# Autodesk Inventor assembly: Manipulator
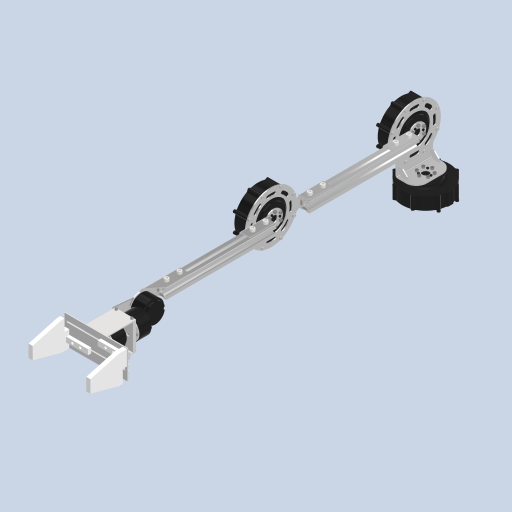
[picture p0: Inventor's stored thumbnail of the model, 512x512]
Saved by Autodesk Inventor 2023 (Build 270158000, 158)
## iProperties
Created: 2024-11-08
Part Number: Manipulator
Document SubType Name: Assembly
Designer: kiyo
Author: kiyo
## Documents named in this file (19)
- D:\GitHub\inventor\syu-si\OfficeRobot\Manipulator\Manipulator.iam
- D:\GitHub\inventor\syu-si\OfficeRobot\ReadyMade\Steadywin\GIM8108-8.iam
- D:\GitHub\inventor\syu-si\OfficeRobot\Manipulator\elbow-pitch-bracket.ipt
- D:\GitHub\inventor\syu-si\OfficeRobot\ReadyMade\Screw\M3_6mm.ipt
- D:\GitHub\inventor\syu-si\OfficeRobot\ReadyMade\Steadywin\GIM3505-8_with-driver.ipt
- D:\GitHub\inventor\syu-si\OfficeRobot\Manipulator\wrist_roll_plate.ipt
- D:\GitHub\inventor\syu-si\OfficeRobot\Manipulator\wrist-pitch-plate.ipt
- D:\GitHub\inventor\syu-si\OfficeRobot\ReadyMade\Screw\M2-5_6mm.ipt
- D:\GitHub\inventor\syu-si\OfficeRobot\ReadyMade\Screw\CBSH3-8.ipt
- D:\GitHub\inventor\syu-si\OfficeRobot\ReadyMade\Screw\FWSJJ-D5-V2_6-T4_5.ipt
- D:\GitHub\inventor\syu-si\OfficeRobot\ReadyMade\Screw\M2-5_10mm.ipt
- D:\GitHub\inventor\syu-si\OfficeRobot\ReadyMade\Screw\HNTU5-5.ipt
- D:\GitHub\inventor\syu-si\OfficeRobot\Manipulator\pitch_plate_20mm.ipt
- D:\GitHub\inventor\syu-si\OfficeRobot\ReadyMade\Aluminum-frame\HFS5-2020-210-AV10-BV35-CV175-DV200.ipt
- D:\GitHub\inventor\syu-si\OfficeRobot\Manipulator\sholder_roll_bracket.ipt
- D:\GitHub\inventor\syu-si\OfficeRobot\ReadyMade\Screw\SCB5-22.ipt
- D:\GitHub\inventor\syu-si\OfficeRobot\ReadyMade\Screw\SCB5-8.ipt
- D:\GitHub\inventor\syu-si\OfficeRobot\Manipulator\Hand_tyokudou.iam
- D:\GitHub\inventor\syu-si\OfficeRobot\ReadyMade\Screw\PACK-SWSJJ10-6-0_3.ipt
## Components (110 placed, 18 different names)
1. pitch_plate_20mm:1 — メイト:3, フラッシュ:1, 挿入:355, 挿入:356, 挿入:357, 挿入:358, 挿入:359, 挿入:360, 角度:47
2. pitch_plate_20mm:2 — 挿入:345, フラッシュ:3, 角度:40
3. elbow-pitch-bracket:1 — 挿入:341, 挿入:342, フラッシュ:2, フラッシュ:7, フラッシュ:8
4. sholder_roll_bracket:1 — 挿入:350, 挿入:361, 挿入:362, 挿入:363, 挿入:364, 挿入:365, 挿入:366, 挿入:414, 挿入:415
5. HFS5-2020-210-AV10-BV35-CV175-DV200:1 — メイト:3, フラッシュ:1, フラッシュ:2, メイト:19, メイト:20, 角度:35, 角度:36, メイト:21, メイト:22, フラッシュ:9, 角度:37, メイト:23, メイト:24
6. HFS5-2020-210-AV10-BV35-CV175-DV200:2 — フラッシュ:3, 挿入:351, 挿入:352, 角度:27, 角度:28, 挿入:353, 挿入:354, 角度:29, 角度:30, メイト:15, メイト:16, 角度:33, フラッシュ:5, メイト:17, メイト:18, 角度:34, フラッシュ:6, メイト:25, メイト:26, メイト:27, メイト:28, メイト:29, メイト:30
7. wrist-pitch-plate:1 — 挿入:409, 挿入:410, メイト:29, メイト:30, 正接:1, 正接:2, 正接:3, 挿入:437, 挿入:438, 挿入:439
8. wrist_roll_plate:2 — 挿入:402, 挿入:403, 挿入:404, 挿入:405, 挿入:406, 挿入:407, 挿入:408
9. Hand_tyokudou:1 [sub-assembly] — 角度:45, 挿入:431, 挿入:434, 挿入:435, 挿入:436
10. PACK-SWSJJ10-6-0_3:1 — 挿入:429
11. PACK-SWSJJ10-6-0_3:2 — 挿入:428
12. PACK-SWSJJ10-6-0_3:3 — 挿入:418
13. PACK-SWSJJ10-6-0_3:4 — 挿入:419
14. PACK-SWSJJ10-6-0_3:5 — 挿入:421
15. PACK-SWSJJ10-6-0_3:6 — 挿入:426
16. PACK-SWSJJ10-6-0_3:7 — 挿入:423
17. PACK-SWSJJ10-6-0_3:8 — 挿入:424
18. PACK-SWSJJ10-6-0_3:9 — 挿入:422
19. PACK-SWSJJ10-6-0_3:10 — 挿入:425
20. PACK-SWSJJ10-6-0_3:11 — 挿入:420
21. PACK-SWSJJ10-6-0_3:12 — 挿入:427
22. PACK-SWSJJ10-6-0_3:13 — 挿入:417
23. PACK-SWSJJ10-6-0_3:14 — 挿入:416
24. FWSJJ-D5-V2_6-T4_5:13 — 挿入:430, 挿入:431
25. M2-5_10mm:10 — 挿入:430
26. FWSJJ-D5-V2_6-T4_5:14 — 挿入:434
27. M2-5_10mm:11
28. FWSJJ-D5-V2_6-T4_5:15 — 挿入:435
29. M2-5_10mm:12
30. M2-5_6mm:16 — 挿入:439
31. M2-5_6mm:17 — 挿入:438
32. M2-5_6mm:18 — 挿入:437
33. M3_6mm:7 — 挿入:337
34. M3_6mm:8 — 挿入:336
35. M3_6mm:9 — 挿入:334
36. M3_6mm:10 — 挿入:338
37. M3_6mm:11 — 挿入:339
38. M3_6mm:12 — 挿入:335
39. M3_6mm:19 — 挿入:358
40. M3_6mm:20 — 挿入:357
41. M3_6mm:21 — 挿入:355
42. M3_6mm:22 — 挿入:356
43. M3_6mm:23 — 挿入:359
44. M3_6mm:24 — 挿入:360
45. M3_6mm:25 — 挿入:361
46. M3_6mm:26 — 挿入:363
47. M3_6mm:27 — 挿入:362
48. M3_6mm:28 — 挿入:364
49. M3_6mm:29 — 挿入:365
50. M3_6mm:30 — 挿入:366
51. CBSH3-8:1 — 挿入:307
52. CBSH3-8:2 — 挿入:308
53. CBSH3-8:3 — 挿入:302
54. CBSH3-8:4 — 挿入:304, 挿入:415
55. CBSH3-8:5 — 挿入:309
56. CBSH3-8:6 — 挿入:303
57. CBSH3-8:7 — 挿入:305
58. CBSH3-8:8 — 挿入:306
59. CBSH3-8:9 — 挿入:332
60. CBSH3-8:10 — 挿入:327
61. CBSH3-8:11 — 挿入:330
62. CBSH3-8:12 — 挿入:328
63. CBSH3-8:13 — 挿入:329
64. CBSH3-8:14 — 挿入:331
65. CBSH3-8:15 — 挿入:326
66. CBSH3-8:16 — 挿入:333
67. M2-5_6mm:13
68. M2-5_6mm:14
69. M2-5_6mm:15
70. M2-5_10mm:7 — 挿入:402
71. M2-5_10mm:8 — 挿入:403
72. M2-5_10mm:9 — 挿入:404
73. FWSJJ-D5-V2_6-T4_5:10 — 挿入:407
74. FWSJJ-D5-V2_6-T4_5:11 — 挿入:405
75. FWSJJ-D5-V2_6-T4_5:12 — 挿入:406
76. HNTU5-5:22 — 挿入:412, メイト:27, メイト:28
77. SCB5-8:8 — 挿入:412, 正接:2, 挿入:429
78. HNTU5-5:23 — 挿入:411, メイト:25, メイト:26
79. SCB5-8:9 — 挿入:411, 正接:3, 挿入:428
80. SCB5-22:1 — 挿入:368, 挿入:418
81. SCB5-22:2 — 挿入:367, 挿入:419
82. SCB5-22:3 — 挿入:370, 挿入:421
83. SCB5-22:4 — 挿入:369, 挿入:420
84. SCB5-22:5 — 挿入:372, 挿入:423
85. SCB5-22:6 — 挿入:371, 挿入:422
86. SCB5-22:7 — 挿入:376, 挿入:416
87. SCB5-22:8 — 挿入:375, 正接:1, 挿入:417
88. SCB5-8:3 — 挿入:427
89. SCB5-8:4
90. SCB5-8:5 — 挿入:426
91. SCB5-8:6 — 挿入:425
92. SCB5-8:7 — 挿入:424
93. HNTU5-5:6 — 挿入:372
94. HNTU5-5:7 — 挿入:371
95. HNTU5-5:9 — 挿入:369
96. HNTU5-5:10 — 挿入:370
97. HNTU5-5:11 — 挿入:351, 角度:28, 挿入:367
98. HNTU5-5:12 — 挿入:352, 角度:27, 挿入:368
99. HNTU5-5:13 — 挿入:353, 角度:30, 挿入:376
100. HNTU5-5:14 — 挿入:354, 角度:29, 挿入:375
101. HNTU5-5:17 — メイト:15, メイト:16, 角度:33, フラッシュ:5
102. HNTU5-5:18 — メイト:17, メイト:18, 角度:34, フラッシュ:6
103. HNTU5-5:19 — フラッシュ:8, メイト:19, メイト:20, 角度:35
104. HNTU5-5:20 — フラッシュ:7, 角度:36, メイト:21, メイト:22
105. HNTU5-5:21 — フラッシュ:9, 角度:37, メイト:23, メイト:24
106. GIM8108-8:1 [sub-assembly] — 挿入:350, 角度:46, 角度:48
107. GIM8108-8:2 [sub-assembly] — 挿入:302, 挿入:303, 挿入:304, 挿入:305, 挿入:306, 挿入:307, 挿入:308, 挿入:309, 角度:46, 挿入:414, 角度:47
108. GIM8108-8:3 [sub-assembly] — 挿入:326, 挿入:327, 挿入:328, 挿入:329, 挿入:330, 挿入:331, 挿入:332, 挿入:333, 挿入:334, 挿入:335, 挿入:336, 挿入:337, 挿入:338, 挿入:339, 挿入:341, 挿入:342, 挿入:345, 角度:40
109. GIM3505-8_with-driver:9 — 挿入:408, 挿入:409, 挿入:410, 角度:44
110. GIM3505-8_with-driver:8 — 角度:44, 角度:45, 挿入:436
## Relationships (155: Insert 102, Mate 22, Angle 20, Flush 8, Tangent 3)
- 挿入:302 [Insert] (2 mm): CBSH3-8:3 ↔ GIM8108-8:2
- 挿入:303 [Insert] (2 mm): CBSH3-8:6 ↔ GIM8108-8:2
- 挿入:304 [Insert] (2 mm): CBSH3-8:4 ↔ GIM8108-8:2
- 挿入:305 [Insert] (2 mm): CBSH3-8:7 ↔ GIM8108-8:2
- 挿入:306 [Insert] (2 mm): CBSH3-8:8 ↔ GIM8108-8:2
- 挿入:307 [Insert] (2 mm): CBSH3-8:1 ↔ GIM8108-8:2
- 挿入:308 [Insert] (2 mm): CBSH3-8:2 ↔ GIM8108-8:2
- 挿入:309 [Insert] (2 mm): CBSH3-8:5 ↔ GIM8108-8:2
- [Insert] (-0.75 mm): HFS5-2020-210-AV10-BV35-CV175-DV200:1 ↔ HNTU5-5:6
- [Angle] (0 deg): HFS5-2020-210-AV10-BV35-CV175-DV200:1 ↔ HNTU5-5:6
- [Insert] (-0.75 mm): HFS5-2020-210-AV10-BV35-CV175-DV200:1 ↔ HNTU5-5:7
- [Angle] (0 deg): HFS5-2020-210-AV10-BV35-CV175-DV200:1 ↔ HNTU5-5:7
- [Angle] (0 deg): HFS5-2020-210-AV10-BV35-CV175-DV200:1 ↔ HNTU5-5:6
- 挿入:326 [Insert] (2 mm): CBSH3-8:15 ↔ GIM8108-8:3
- 挿入:327 [Insert] (2 mm): CBSH3-8:10 ↔ GIM8108-8:3
- 挿入:328 [Insert] (2 mm): CBSH3-8:12 ↔ GIM8108-8:3
- 挿入:329 [Insert] (2 mm): CBSH3-8:13 ↔ GIM8108-8:3
- 挿入:330 [Insert] (2 mm): CBSH3-8:11 ↔ GIM8108-8:3
- 挿入:331 [Insert] (2 mm): CBSH3-8:14 ↔ GIM8108-8:3
- 挿入:332 [Insert] (2 mm): CBSH3-8:9 ↔ GIM8108-8:3
- 挿入:333 [Insert] (2 mm): CBSH3-8:16 ↔ GIM8108-8:3
- 挿入:334 [Insert] (2 mm): M3_6mm:9 ↔ GIM8108-8:3
- 挿入:335 [Insert] (2 mm): M3_6mm:12 ↔ GIM8108-8:3
- 挿入:336 [Insert] (2 mm): M3_6mm:8 ↔ GIM8108-8:3
- 挿入:337 [Insert] (2 mm): M3_6mm:7 ↔ GIM8108-8:3
- 挿入:338 [Insert] (2 mm): M3_6mm:10 ↔ GIM8108-8:3
- 挿入:339 [Insert] (2 mm): M3_6mm:11 ↔ GIM8108-8:3
- [Insert]: pitch_plate_20mm:1 ↔ GIM8108-8:2
- [Mate] (0.3 mm): pitch_plate_20mm:1 ↔ HFS5-2020-210-AV10-BV35-CV175-DV200:1
- メイト:3 [Mate] (0.3 mm): pitch_plate_20mm:1 ↔ HFS5-2020-210-AV10-BV35-CV175-DV200:1
- 挿入:341 [Insert]: elbow-pitch-bracket:1 ↔ GIM8108-8:3
- 挿入:342 [Insert]: elbow-pitch-bracket:1 ↔ GIM8108-8:3
- [Angle] (0 deg): HFS5-2020-210-AV10-BV35-CV175-DV200:1 ↔ HNTU5-5:9
- [Angle] (0 deg): HFS5-2020-210-AV10-BV35-CV175-DV200:1 ↔ HNTU5-5:10
- [Insert] (-0.75 mm): HFS5-2020-210-AV10-BV35-CV175-DV200:1 ↔ HNTU5-5:9
- [Insert] (-0.75 mm): HFS5-2020-210-AV10-BV35-CV175-DV200:1 ↔ HNTU5-5:10
- [Mate] (0.3 mm): elbow-pitch-bracket:1 ↔ HFS5-2020-210-AV10-BV35-CV175-DV200:1
- [Mate] (0.3 mm): elbow-pitch-bracket:1 ↔ HFS5-2020-210-AV10-BV35-CV175-DV200:1
- 挿入:345 [Insert]: pitch_plate_20mm:2 ↔ GIM8108-8:3
- [Mate] (0.3 mm): pitch_plate_20mm:2 ↔ HFS5-2020-210-AV10-BV35-CV175-DV200:2
- [Mate] (0.3 mm): pitch_plate_20mm:2 ↔ HFS5-2020-210-AV10-BV35-CV175-DV200:2
- 挿入:350 [Insert]: sholder_roll_bracket:1 ↔ GIM8108-8:1
- フラッシュ:1 [Flush]: pitch_plate_20mm:1 ↔ HFS5-2020-210-AV10-BV35-CV175-DV200:1
- フラッシュ:2 [Flush]: elbow-pitch-bracket:1 ↔ HFS5-2020-210-AV10-BV35-CV175-DV200:1
- フラッシュ:3 [Flush]: pitch_plate_20mm:2 ↔ HFS5-2020-210-AV10-BV35-CV175-DV200:2
- 挿入:351 [Insert] (-0.75 mm): HFS5-2020-210-AV10-BV35-CV175-DV200:2 ↔ HNTU5-5:11
- 挿入:352 [Insert] (-0.75 mm): HFS5-2020-210-AV10-BV35-CV175-DV200:2 ↔ HNTU5-5:12
- 角度:27 [Angle] (0 deg): HFS5-2020-210-AV10-BV35-CV175-DV200:2 ↔ HNTU5-5:12
- 角度:28 [Angle] (0 deg): HFS5-2020-210-AV10-BV35-CV175-DV200:2 ↔ HNTU5-5:11
- 挿入:353 [Insert] (-0.75 mm): HFS5-2020-210-AV10-BV35-CV175-DV200:2 ↔ HNTU5-5:13
- 挿入:354 [Insert] (-0.75 mm): HFS5-2020-210-AV10-BV35-CV175-DV200:2 ↔ HNTU5-5:14
- 角度:29 [Angle] (0 deg): HFS5-2020-210-AV10-BV35-CV175-DV200:2 ↔ HNTU5-5:14
- 角度:30 [Angle] (0 deg): HFS5-2020-210-AV10-BV35-CV175-DV200:2 ↔ HNTU5-5:13
- 挿入:355 [Insert]: pitch_plate_20mm:1 ↔ M3_6mm:21
- 挿入:356 [Insert]: pitch_plate_20mm:1 ↔ M3_6mm:22
- 挿入:357 [Insert]: pitch_plate_20mm:1 ↔ M3_6mm:20
- 挿入:358 [Insert]: pitch_plate_20mm:1 ↔ M3_6mm:19
- 挿入:359 [Insert]: pitch_plate_20mm:1 ↔ M3_6mm:23
- 挿入:360 [Insert]: pitch_plate_20mm:1 ↔ M3_6mm:24
- 挿入:361 [Insert]: sholder_roll_bracket:1 ↔ M3_6mm:25
- 挿入:362 [Insert]: sholder_roll_bracket:1 ↔ M3_6mm:27
- 挿入:363 [Insert]: sholder_roll_bracket:1 ↔ M3_6mm:26
- 挿入:364 [Insert]: sholder_roll_bracket:1 ↔ M3_6mm:28
- 挿入:365 [Insert]: sholder_roll_bracket:1 ↔ M3_6mm:29
- 挿入:366 [Insert]: sholder_roll_bracket:1 ↔ M3_6mm:30
- 挿入:367 [Insert] (-0.95 mm): SCB5-22:2 ↔ HNTU5-5:11
- 挿入:368 [Insert] (-0.95 mm): SCB5-22:1 ↔ HNTU5-5:12
- 挿入:369 [Insert] (-0.95 mm): SCB5-22:4 ↔ HNTU5-5:9
- 挿入:370 [Insert] (-0.95 mm): SCB5-22:3 ↔ HNTU5-5:10
- 挿入:371 [Insert] (-0.95 mm): SCB5-22:6 ↔ HNTU5-5:7
- 挿入:372 [Insert] (-0.95 mm): SCB5-22:5 ↔ HNTU5-5:6
- 挿入:375 [Insert] (-0.95 mm): SCB5-22:8 ↔ HNTU5-5:14
- 挿入:376 [Insert] (-0.95 mm): SCB5-22:7 ↔ HNTU5-5:13
- [Insert] (3.5 mm): SCB5-8:3 ↔ HNTU5-5:17
- メイト:15 [Mate]: HFS5-2020-210-AV10-BV35-CV175-DV200:2 ↔ HNTU5-5:17
- メイト:16 [Mate] (1 mm): HFS5-2020-210-AV10-BV35-CV175-DV200:2 ↔ HNTU5-5:17
- 角度:33 [Angle] (0 deg): HFS5-2020-210-AV10-BV35-CV175-DV200:2 ↔ HNTU5-5:17
- フラッシュ:5 [Flush] (33.5 mm): HFS5-2020-210-AV10-BV35-CV175-DV200:2 ↔ HNTU5-5:17
- [Insert] (3.2 mm): SCB5-8:4 ↔ HNTU5-5:18
- メイト:17 [Mate]: HFS5-2020-210-AV10-BV35-CV175-DV200:2 ↔ HNTU5-5:18
- メイト:18 [Mate] (1 mm): HFS5-2020-210-AV10-BV35-CV175-DV200:2 ↔ HNTU5-5:18
- 角度:34 [Angle] (0 deg): HFS5-2020-210-AV10-BV35-CV175-DV200:2 ↔ HNTU5-5:18
- フラッシュ:6 [Flush] (33.5 mm): HFS5-2020-210-AV10-BV35-CV175-DV200:2 ↔ HNTU5-5:18
- [Insert] (3.5 mm): SCB5-8:5 ↔ HNTU5-5:19
- [Insert] (3.5 mm): SCB5-8:6 ↔ HNTU5-5:20
- フラッシュ:7 [Flush] (5.5 mm): elbow-pitch-bracket:1 ↔ HNTU5-5:20
- フラッシュ:8 [Flush] (-30.5 mm): elbow-pitch-bracket:1 ↔ HNTU5-5:19
- メイト:19 [Mate]: HFS5-2020-210-AV10-BV35-CV175-DV200:1 ↔ HNTU5-5:19
- メイト:20 [Mate] (1 mm): HFS5-2020-210-AV10-BV35-CV175-DV200:1 ↔ HNTU5-5:19
- 角度:35 [Angle] (0 deg): HFS5-2020-210-AV10-BV35-CV175-DV200:1 ↔ HNTU5-5:19
- 角度:36 [Angle] (0 deg): HFS5-2020-210-AV10-BV35-CV175-DV200:1 ↔ HNTU5-5:20
- メイト:21 [Mate] (1 mm): HFS5-2020-210-AV10-BV35-CV175-DV200:1 ↔ HNTU5-5:20
- メイト:22 [Mate]: HFS5-2020-210-AV10-BV35-CV175-DV200:1 ↔ HNTU5-5:20
- [Insert] (3.5 mm): SCB5-8:7 ↔ HNTU5-5:21
- フラッシュ:9 [Flush] (33.5 mm): HFS5-2020-210-AV10-BV35-CV175-DV200:1 ↔ HNTU5-5:21
- 角度:37 [Angle] (0 deg): HFS5-2020-210-AV10-BV35-CV175-DV200:1 ↔ HNTU5-5:21
- メイト:23 [Mate] (1 mm): HFS5-2020-210-AV10-BV35-CV175-DV200:1 ↔ HNTU5-5:21
- メイト:24 [Mate]: HFS5-2020-210-AV10-BV35-CV175-DV200:1 ↔ HNTU5-5:21
- 角度:40 [Angle] (0 deg): pitch_plate_20mm:2 ↔ GIM8108-8:3
- [Insert]: wrist_roll_plate:2 ↔ M2-5_6mm:13
- [Insert]: wrist_roll_plate:2 ↔ M2-5_6mm:14
- [Insert]: wrist_roll_plate:2 ↔ M2-5_6mm:15
- [Insert]: wrist_roll_plate:2 ↔ GIM3505-8_with-driver:8
- [Insert]: wrist_roll_plate:2 ↔ GIM3505-8_with-driver:8
- 挿入:402 [Insert]: wrist_roll_plate:2 ↔ M2-5_10mm:7
- 挿入:403 [Insert]: wrist_roll_plate:2 ↔ M2-5_10mm:8
- 挿入:404 [Insert]: wrist_roll_plate:2 ↔ M2-5_10mm:9
- 挿入:405 [Insert]: wrist_roll_plate:2 ↔ FWSJJ-D5-V2_6-T4_5:11
- 挿入:406 [Insert]: wrist_roll_plate:2 ↔ FWSJJ-D5-V2_6-T4_5:12
- 挿入:407 [Insert]: wrist_roll_plate:2 ↔ FWSJJ-D5-V2_6-T4_5:10
- 挿入:408 [Insert] (3.5 mm): wrist_roll_plate:2 ↔ GIM3505-8_with-driver:9
- 挿入:409 [Insert]: wrist-pitch-plate:1 ↔ GIM3505-8_with-driver:9
- 挿入:410 [Insert]: wrist-pitch-plate:1 ↔ GIM3505-8_with-driver:9
- 挿入:411 [Insert] (3.5 mm): HNTU5-5:23 ↔ SCB5-8:9
- 挿入:412 [Insert] (3.5 mm): HNTU5-5:22 ↔ SCB5-8:8
- メイト:25 [Mate]: HFS5-2020-210-AV10-BV35-CV175-DV200:2 ↔ HNTU5-5:23
- メイト:26 [Mate] (1 mm): HFS5-2020-210-AV10-BV35-CV175-DV200:2 ↔ HNTU5-5:23
- メイト:27 [Mate] (1 mm): HFS5-2020-210-AV10-BV35-CV175-DV200:2 ↔ HNTU5-5:22
- メイト:28 [Mate]: HFS5-2020-210-AV10-BV35-CV175-DV200:2 ↔ HNTU5-5:22
- メイト:29 [Mate] (0.3 mm): HFS5-2020-210-AV10-BV35-CV175-DV200:2 ↔ wrist-pitch-plate:1
- メイト:30 [Mate] (0.3 mm): HFS5-2020-210-AV10-BV35-CV175-DV200:2 ↔ wrist-pitch-plate:1
- 正接:1 [Tangent] (0.25 mm): wrist-pitch-plate:1 ↔ SCB5-22:8
- 正接:2 [Tangent] (0.25 mm): wrist-pitch-plate:1 ↔ SCB5-8:8
- 正接:3 [Tangent] (0.25 mm): wrist-pitch-plate:1 ↔ SCB5-8:9
- 角度:44 [Angle] (0 deg): GIM3505-8_with-driver:9 ↔ GIM3505-8_with-driver:8
- 角度:45 [Angle] (0 deg): Hand_tyokudou:1 ↔ GIM3505-8_with-driver:8
- 角度:46 [Angle] (0 deg): GIM8108-8:1 ↔ GIM8108-8:2
- 挿入:414 [Insert]: sholder_roll_bracket:1 ↔ GIM8108-8:2
- 挿入:415 [Insert]: sholder_roll_bracket:1 ↔ CBSH3-8:4
- 角度:47 [Angle] (0 deg): pitch_plate_20mm:1 ↔ GIM8108-8:2
- 角度:48 [Angle] (0 deg): GIM8108-8:1
- 挿入:416 [Insert] (2 mm): PACK-SWSJJ10-6-0_3:14 ↔ SCB5-22:7
- 挿入:417 [Insert] (2 mm): PACK-SWSJJ10-6-0_3:13 ↔ SCB5-22:8
- 挿入:418 [Insert] (2 mm): PACK-SWSJJ10-6-0_3:3 ↔ SCB5-22:1
- 挿入:419 [Insert] (2 mm): PACK-SWSJJ10-6-0_3:4 ↔ SCB5-22:2
- 挿入:420 [Insert] (2 mm): PACK-SWSJJ10-6-0_3:11 ↔ SCB5-22:4
- 挿入:421 [Insert] (2 mm): PACK-SWSJJ10-6-0_3:5 ↔ SCB5-22:3
- 挿入:422 [Insert] (2 mm): PACK-SWSJJ10-6-0_3:9 ↔ SCB5-22:6
- 挿入:423 [Insert] (2 mm): PACK-SWSJJ10-6-0_3:7 ↔ SCB5-22:5
- 挿入:424 [Insert] (2 mm): PACK-SWSJJ10-6-0_3:8 ↔ SCB5-8:7
- 挿入:425 [Insert] (2 mm): PACK-SWSJJ10-6-0_3:10 ↔ SCB5-8:6
- 挿入:426 [Insert] (2 mm): PACK-SWSJJ10-6-0_3:6 ↔ SCB5-8:5
- 挿入:427 [Insert] (2 mm): PACK-SWSJJ10-6-0_3:12 ↔ SCB5-8:3
- 挿入:428 [Insert] (2 mm): PACK-SWSJJ10-6-0_3:2 ↔ SCB5-8:9
- 挿入:429 [Insert] (2 mm): PACK-SWSJJ10-6-0_3:1 ↔ SCB5-8:8
- 挿入:430 [Insert] (2 mm): FWSJJ-D5-V2_6-T4_5:13 ↔ M2-5_10mm:10
- 挿入:431 [Insert]: Hand_tyokudou:1 ↔ FWSJJ-D5-V2_6-T4_5:13
- [Insert] (2 mm): FWSJJ-D5-V2_6-T4_5:14 ↔ M2-5_10mm:11
- [Insert] (2 mm): FWSJJ-D5-V2_6-T4_5:15 ↔ M2-5_10mm:12
- 挿入:434 [Insert]: Hand_tyokudou:1 ↔ FWSJJ-D5-V2_6-T4_5:14
- 挿入:435 [Insert]: Hand_tyokudou:1 ↔ FWSJJ-D5-V2_6-T4_5:15
- 挿入:436 [Insert] (4.5 mm): Hand_tyokudou:1 ↔ GIM3505-8_with-driver:8
- 挿入:437 [Insert]: wrist-pitch-plate:1 ↔ M2-5_6mm:18
- 挿入:438 [Insert]: wrist-pitch-plate:1 ↔ M2-5_6mm:17
- 挿入:439 [Insert]: wrist-pitch-plate:1 ↔ M2-5_6mm:16
## Named parameters: d472_d466 = 3.5 mm, d477_d466 = 3.2 mm, d482_d466 = 3.5 mm, d483_d466 = 3.5 mm, d492_d466 = 3.5 mm, d516_d512 = 0 mm, d517_d513 = 0 mm, d519_d268 = 0 mm, d520_d269 = 0 mm, d521_d270 = 0 mm, d583_d581 = 2 mm, d584_d581 = 2 mm
